# Autodesk Inventor assembly: czlon_2
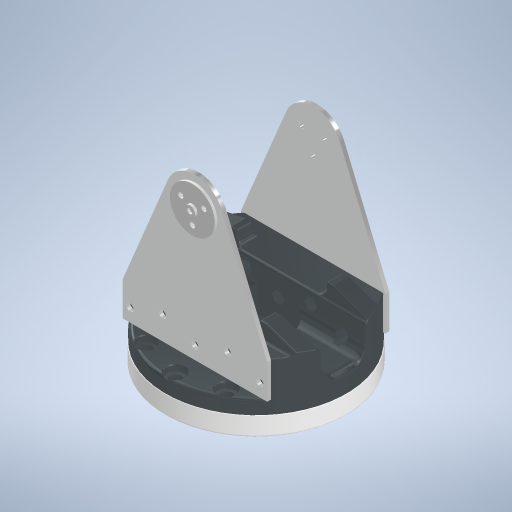
[picture p0: Inventor's stored thumbnail of the model, 512x512]
Saved by Autodesk Inventor 2023 (Build 270158000, 158)
## iProperties
Created: 2023-04-11
Part Number: czlon_2
Document SubType Name: Assembly
Designer: Kamil
Author: Kamil
## Documents named in this file (5)
- C:\Users\Kamil\Desktop\KONARM_2\czlon 2\czlon_2.iam
- C:\Users\Kamil\Desktop\KONARM_2\czlon 2\BLACHA_2_Przegub.ipt
- C:\Users\Kamil\Desktop\KONARM_2\czlon 2\lacznik_kopia.ipt
- C:\Users\Kamil\Desktop\KONARM_2\czlon 2\Góra.ipt
- C:\Users\Kamil\Desktop\KONARM_2\czlon 2\na magnes.ipt
## Components (5 placed, 4 different names)
1. BLACHA_2_Przegub:1 — Zestawiające:4, Zestawiające:5, Zestawiające:6, Zestawiające:9, Zestawiające:10, Zestawiające:11
2. lacznik_kopia:1 — Zestawiające:1, Zestawiające:2, Zestawiające:3, Zestawiające:4, Zestawiające:5, Zestawiające:6, Zestawiające:7, Zestawiające:8
3. Góra:1 — Zestawiające:1, Zestawiające:2
4. BLACHA_2_Przegub:2 — Zestawiające:3, Zestawiające:7, Zestawiające:8
5. na magnes:2 — Zestawiające:9, Zestawiające:10, Zestawiające:11
## Relationships (11: Mate 11)
- Zestawiające:1 [Mate]: lacznik_kopia:1 ↔ Góra:1
- Zestawiające:2 [Mate]: lacznik_kopia:1 ↔ Góra:1
- Zestawiające:3 [Mate]: lacznik_kopia:1 ↔ BLACHA_2_Przegub:2
- Zestawiające:4 [Mate]: BLACHA_2_Przegub:1 ↔ lacznik_kopia:1
- Zestawiające:5 [Mate]: BLACHA_2_Przegub:1 ↔ lacznik_kopia:1
- Zestawiające:6 [Mate]: BLACHA_2_Przegub:1 ↔ lacznik_kopia:1
- Zestawiające:7 [Mate]: lacznik_kopia:1 ↔ BLACHA_2_Przegub:2
- Zestawiające:8 [Mate]: lacznik_kopia:1 ↔ BLACHA_2_Przegub:2
- Zestawiające:9 [Mate]: BLACHA_2_Przegub:1 ↔ na magnes:2
- Zestawiające:10 [Mate]: BLACHA_2_Przegub:1 ↔ na magnes:2
- Zestawiające:11 [Mate]: BLACHA_2_Przegub:1 ↔ na magnes:2
